# Autodesk Inventor assembly: DribblerUnit
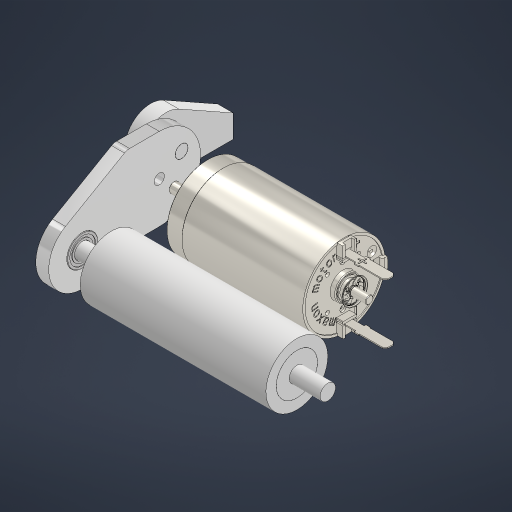
[picture p0: Inventor's stored thumbnail of the model, 512x512]
Saved by Autodesk Inventor 2024.2 (Build 282272000, 272)
## iProperties
Created: 2023-12-27
Part Number: DribblerUnit
Document SubType Name: Assembly
Designer: Hanaoka
Author: Hanaoka
## Documents named in this file (10)
- G:\共有ドライブ\reRo\05_個人\hanaoka\inventor\DribblerUnit\DribblerUnit.iam
- G:\共有ドライブ\reRo\05_個人\hanaoka\inventor\DribblerUnit\Dribbler_Tube.ipt
- G:\共有ドライブ\reRo\05_個人\hanaoka\inventor\DribblerUnit\Shaft_350.ipt
- G:\共有ドライブ\reRo\05_個人\hanaoka\inventor\DribblerUnit\Bearing_C-FL673ZZ\Bearing_C-FL673ZZ.ipt
- G:\共有ドライブ\reRo\05_個人\hanaoka\inventor\DribblerUnit\Tube_Hub.ipt
- G:\共有ドライブ\reRo\05_個人\hanaoka\inventor\HandleUnit\GearCover.ipt
- G:\共有ドライブ\reRo\05_個人\hanaoka\inventor\Stand.ipt
- G:\共有ドライブ\reRo\05_個人\hanaoka\inventor\DribblerUnit\Bearing_C-SFL682AZZ\Bearing_C-SFL682AZZ.ipt
- G:\共有ドライブ\reRo\05_個人\hanaoka\inventor\NockPin_2.5x6.ipt
- G:\共有ドライブ\reRo\05_個人\hanaoka\inventor\DribblerUnit\0_1\dcx16s.iam
## Components (9 placed, 9 different names)
1. Dribbler_Tube:1 — 挿入:12
2. Shaft_350:1 — 挿入:1, 挿入:13
3. Bearing_C-FL673ZZ:1 — 挿入:1, 挿入:6
4. Tube_Hub:1 — 挿入:12, 挿入:13
5. GearCover:1 — 挿入:6, 挿入:14
6. Stand:1 — 挿入:15
7. Bearing_C-SFL682AZZ:1 — 挿入:15, 挿入:16
8. NockPin_2.5x6:1 — 挿入:14, 挿入:16
9. dcx16s:1 [sub-assembly]
## Relationships (7: Insert 7)
- 挿入:1 [Insert]: Shaft_350:1 ↔ Bearing_C-FL673ZZ:1
- 挿入:6 [Insert]: Bearing_C-FL673ZZ:1 ↔ GearCover:1
- 挿入:12 [Insert]: Dribbler_Tube:1 ↔ Tube_Hub:1
- 挿入:13 [Insert] (8 mm): Shaft_350:1 ↔ Tube_Hub:1
- 挿入:14 [Insert]: GearCover:1 ↔ NockPin_2.5x6:1
- 挿入:15 [Insert]: Stand:1 ↔ Bearing_C-SFL682AZZ:1
- 挿入:16 [Insert]: Bearing_C-SFL682AZZ:1 ↔ NockPin_2.5x6:1
